# Autodesk Inventor assembly: lw_5_сборка
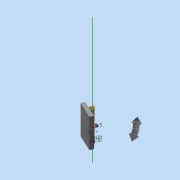
[picture p0: Inventor's stored thumbnail of the model, 180x180]
Saved by Autodesk Inventor 2019 (Build 230136000, 136)
## iProperties
Created: 2021-05-08
Part Number: lw_5_сборка
Material: Типовые
Document SubType Name: Assembly
Designer: Kurbatova
Author: Kurbatova
## Documents named in this file (3)
- C:\Users\Kurbatova\source\LW2021\LW_SAPR\Сборки\lw_5_сборка.iam
- C:\Users\Kurbatova\source\LW2021\LW_SAPR\Детали\lw_5_цилиндр.ipt
- C:\Users\Kurbatova\source\LW2021\LW_SAPR\Детали\lw_5_корпус_new.ipt
## Components (2 placed, 2 different names)
1. lw_5_корпус_new:1 — Совмещение:1, Заподлицо:1
2. lw_5_цилиндр:1 — Совмещение:1, Заподлицо:1
## Relationships (2: Mate 1, Flush 1)
- Совмещение:1 [Mate]: lw_5_корпус_new:1 ↔ lw_5_цилиндр:1
- Заподлицо:1 [Flush]: lw_5_корпус_new:1 ↔ lw_5_цилиндр:1
